# Autodesk Inventor assembly: auger_assembly
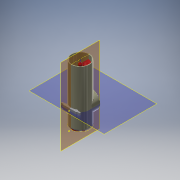
[picture p0: Inventor's stored thumbnail of the model, 180x180]
Saved by Autodesk Inventor 2019 (Build 230136000, 136)
## iProperties
Created: 2019-05-05
Part Number: auger_assembly
Document SubType Name: Assembly
Designer: assman
Author: assman
## Documents named in this file (4)
- D:\Inventor\Projects\CatFeeder\Case\version7\auger_assembly.iam
- D:\Inventor\Projects\CatFeeder\Case\version7\auger_case.ipt
- D:\Inventor\Projects\CatFeeder\Case\version7\auger.ipt
- D:\Inventor\Projects\CatFeeder\Case\version7\motor_support.ipt
## Components (3 placed, 3 different names)
1. auger_case:1 — Flush:1, Flush:2, Rigid:1
2. auger:1 — Flush:1, Flush:2
3. motor_support:1 — Rigid:1
## Relationships (3: Flush 2, WeldJoint 1)
- Flush:1: auger_case:1 ↔ auger:1
- Flush:2: auger_case:1 ↔ auger:1
- Rigid:1 [WeldJoint]: auger_case:1 ↔ motor_support:1
